# Autodesk Inventor assembly: Assembly1
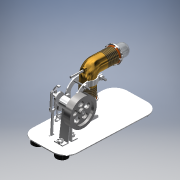
[picture p0: Inventor's stored thumbnail of the model, 180x180]
Saved by Autodesk Inventor 2018 (Build 220112000, 112)
## iProperties
Created: 2018-03-02
Part Number: Assembly1
Document SubType Name: Assembly
Designer: 238438
Author: 238438
## Documents named in this file (27)
- P:\ied\reverso enginero\Assembly1.iam
- P:\ied\reverso enginero\base.ipt
- P:\ied\reverso enginero\ARM.ipt
- P:\ied\reverso enginero\sqrew base.ipt
- P:\ied\reverso enginero\nut for base.ipt
- P:\ied\reverso enginero\baringstand.ipt
- P:\ied\reverso enginero\sqrew for baring stand.ipt
- P:\ied\reverso enginero\bend.ipt
- P:\ied\reverso enginero\srew long.ipt
- P:\ied\reverso enginero\nut for sqrew long.ipt
- P:\ied\reverso enginero\piston rod.ipt
- P:\ied\reverso enginero\baring.ipt
- P:\ied\reverso enginero\fly wheel.ipt
- P:\ied\reverso enginero\piston rod sqrew.ipt
- P:\ied\reverso enginero\piston.ipt
- P:\ied\reverso enginero\piston cup.ipt
- P:\ied\reverso enginero\seal.ipt
- P:\ied\reverso enginero\seal cap.ipt
- P:\ied\reverso enginero\rocker.ipt
- P:\ied\reverso enginero\pin 1.ipt
- P:\ied\reverso enginero\nut for baring.ipt
- P:\ied\reverso enginero\bottun tube.ipt
- P:\ied\reverso enginero\buttom piston.ipt
- P:\ied\reverso enginero\ociy boy.ipt
- P:\ied\reverso enginero\ARM LONG.ipt
- P:\ied\reverso enginero\pin 2.ipt
- P:\ied\reverso enginero\piston holder thing.ipt
## Components (35 placed, 26 different names)
1. base:1 — Mate:1, Mate:2, Mate:6, Mate:7, Mate:8, Mate:9, Flush:3, Mate:39, Mate:41, Mate:50, Flush:9, Mate:62, Mate:63, Flush:12
2. ARM:1 — Mate:1, Mate:2, Mate:3, Mate:4, Mate:12, Flush:3, Flush:4, Mate:13, Mate:14, Mate:15, Mate:16, Mate:18, Mate:20, Mate:35, Flush:7, Mate:37, Mate:58
3. sqrew base:1 — Mate:3, Mate:4, Mate:5
4. nut for base:1 — Mate:5, Mate:6
5. baringstand:1 — Mate:7, Tangent:1, Mate:10, Mate:11, Tangent:2, Tangent:3, Mate:25, Flush:5
6. sqrew for baring stand:1 — Mate:8, Tangent:1, Mate:10, Tangent:2, Mate:40
7. sqrew for baring stand:2 — Mate:9, Mate:11, Tangent:3, Mate:38
8. bend:1 — Mate:12, Flush:4, Mate:29, Mate:30, Mate:31, Mate:32, Mate:33, Mate:34, Mate:43, Mate:44, Flush:8, Mate:46, Mate:47
9. srew long:1 — Mate:13, Mate:14, Mate:17
10. srew long:2 — Mate:15, Mate:16, Mate:19
11. nut for sqrew long:1 — Mate:17, Mate:18
12. nut for sqrew long:2 — Mate:19, Mate:20
13. piston rod:1 — Mate:21, Mate:22, Mate:23, Mate:24, Mate:26, Mate:27, Mate:28, Mate:51, Mate:52, Mate:61
14. baring:1 — Mate:21, Mate:22
15. baring:2 — Mate:23, Mate:24, Mate:25, Flush:5
16. fly wheel:1 — Mate:26, Mate:27, Flush:6
17. piston rod sqrew:1 — Mate:28, Flush:6
18. piston:1 — Mate:29, Mate:30
19. piston cup:1 — Mate:31, Mate:32, Mate:42
20. seal:1 — Mate:42, Mate:43
21. seal cap:1 — Mate:33, Mate:34
22. rocker:1 — Mate:36, Mate:37, Mate:53, Flush:10, Mate:57, Flush:11, Mate:58, Mate:59
23. pin 1:1 — Mate:35, Mate:36, Flush:7, Mate:59
24. nut for baring:1 — Mate:38, Mate:39
25. nut for baring:2 — Mate:40, Mate:41
26. bottun tube:1 — Mate:44, Flush:8, Mate:45
27. buttom piston:1 — Mate:45, Mate:55, Mate:56
28. seal cap:2 — Mate:46, Mate:47, Mate:48, Mate:49
29. seal:2 — Mate:48, Mate:49
30. ociy boy:1 — Mate:50, Flush:9, Mate:61, Mate:62, Mate:64
31. ARM LONG:1 — Mate:51, Mate:52
32. pin 2:1 — Mate:53, Flush:10
33. piston holder thing:1 — Mate:55, Mate:56, Mate:60
34. pin 2:2 — Mate:57, Flush:11, Mate:60
35. pin 2:3 — Mate:63, Flush:12, Mate:64
## Relationships (76: Mate 63, Flush 10, Tangent 3)
- Mate:1: base:1 ↔ ARM:1
- Mate:2: base:1 ↔ ARM:1
- Mate:3: ARM:1 ↔ sqrew base:1
- Mate:4: ARM:1 ↔ sqrew base:1
- Mate:5: sqrew base:1 ↔ nut for base:1
- Mate:6: base:1 ↔ nut for base:1
- Mate:7: base:1 ↔ baringstand:1
- Mate:8: base:1 ↔ sqrew for baring stand:1
- Mate:9: base:1 ↔ sqrew for baring stand:2
- Tangent:1: baringstand:1 ↔ sqrew for baring stand:1
- Mate:10: baringstand:1 ↔ sqrew for baring stand:1
- Mate:11: baringstand:1 ↔ sqrew for baring stand:2
- Tangent:2 (-0.635 mm): baringstand:1 ↔ sqrew for baring stand:1
- Tangent:3: baringstand:1 ↔ sqrew for baring stand:2
- Mate:12: ARM:1 ↔ bend:1
- Flush:3 (13.4874 mm): base:1 ↔ ARM:1
- Flush:4 (17.3736 mm): ARM:1 ↔ bend:1
- Mate:13: ARM:1 ↔ srew long:1
- Mate:14: ARM:1 ↔ srew long:1
- Mate:15: ARM:1 ↔ srew long:2
- Mate:16: ARM:1 ↔ srew long:2
- Mate:17: srew long:1 ↔ nut for sqrew long:1
- Mate:18: ARM:1 ↔ nut for sqrew long:1
- Mate:19: srew long:2 ↔ nut for sqrew long:2
- Mate:20: ARM:1 ↔ nut for sqrew long:2
- Mate:21: piston rod:1 ↔ baring:1
- Mate:22: piston rod:1 ↔ baring:1
- Mate:23: piston rod:1 ↔ baring:2
- Mate:24: piston rod:1 ↔ baring:2
- Mate:25: baringstand:1 ↔ baring:2
- Flush:5: baringstand:1 ↔ baring:2
- Mate:26: piston rod:1 ↔ fly wheel:1
- Mate:27: piston rod:1 ↔ fly wheel:1
- Mate:28: piston rod:1 ↔ piston rod sqrew:1
- Flush:6: fly wheel:1 ↔ piston rod sqrew:1
- Mate:29: bend:1 ↔ piston:1
- Mate:30: bend:1 ↔ piston:1
- Mate:31: bend:1 ↔ piston cup:1
- Mate:32: bend:1 ↔ piston cup:1
- Mate:33: bend:1 ↔ seal cap:1
- Mate:34: bend:1 ↔ seal cap:1
- Mate:35: ARM:1 ↔ pin 1:1
- Mate:36: rocker:1 ↔ pin 1:1
- Flush:7 (-0.635 mm): ARM:1 ↔ pin 1:1
- Mate:37 (0.635 mm): ARM:1 ↔ rocker:1
- Mate:38: sqrew for baring stand:2 ↔ nut for baring:1
- Mate:39: base:1 ↔ nut for baring:1
- Mate:40: sqrew for baring stand:1 ↔ nut for baring:2
- Mate:41: base:1 ↔ nut for baring:2
- Mate:42: piston cup:1 ↔ seal:1
- Mate:43: bend:1 ↔ seal:1
- Mate:44: bend:1 ↔ bottun tube:1
- Flush:8: bend:1 ↔ bottun tube:1
- Mate:45: bottun tube:1 ↔ buttom piston:1
- Mate:46: bend:1 ↔ seal cap:2
- Mate:47: bend:1 ↔ seal cap:2
- Mate:48: seal cap:2 ↔ seal:2
- Mate:49 (-1.27 mm): seal cap:2 ↔ seal:2
- Mate:50 (0.127 mm): base:1 ↔ ociy boy:1
- Flush:9 (1.524 mm): base:1 ↔ ociy boy:1
- Mate:51: piston rod:1 ↔ ARM LONG:1
- Mate:52 (0.127 mm): piston rod:1 ↔ ARM LONG:1
- Mate:53: rocker:1 ↔ pin 2:1
- Flush:10: rocker:1 ↔ pin 2:1
- Mate:55: buttom piston:1 ↔ piston holder thing:1
- Mate:56 (-1.27 mm): buttom piston:1 ↔ piston holder thing:1
- Mate:57: rocker:1 ↔ pin 2:2
- Flush:11: rocker:1 ↔ pin 2:2
- Mate:58 (0.5715 mm): ARM:1 ↔ rocker:1
- Mate:59: rocker:1 ↔ pin 1:1
- Mate:60: piston holder thing:1 ↔ pin 2:2
- Mate:61: piston rod:1 ↔ ociy boy:1
- Mate:62 (2.54 mm): base:1 ↔ ociy boy:1
- Mate:63: base:1 ↔ pin 2:3
- Flush:12: base:1 ↔ pin 2:3
- Mate:64: ociy boy:1 ↔ pin 2:3
